# Autodesk Inventor assembly: MG-Grundplatte
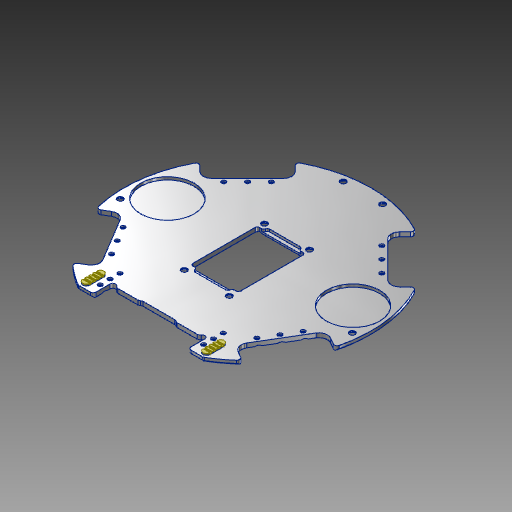
[picture p0: Inventor's stored thumbnail of the model, 512x512]
Saved by Autodesk Inventor 2019.4 (Build 234330000, 330)
## iProperties
Part Number: MG-Grundplatte
Material: Generisch
Document SubType Name: Assembly
Designer: rYan
Mass: 128.652 g
Surface Area: 395.086 cm^2
Volume: 47.6131 cm^3
Density: 2.70203 g/cm^3
Author: rYan
## Documents named in this file (3)
- D:\TIGERsGIT\Hardware\mechanik\2020\Inventor\Robot\MG-Grundplatte.iam
- D:\TIGERsGIT\Hardware\mechanik\2020\Inventor\Robot\Grundplatte.ipt
- D:\TIGERsGIT\Hardware\mechanik\2020\Inventor\Robot\Dribbler\Dribblerdaempfer Unten.ipt
## Components (3 placed, 2 different names)
1. Grundplatte:1 — Fluchtend:1, Passend:1, Passend:2, Passend:3, Passend:4, Tangential:1, Tangential:2, Passend:5, Passend:6
2. Dribblerdaempfer Unten:1 — Passend:3, Tangential:2, Passend:6
3. Dribblerdaempfer Unten:2 — Passend:4, Tangential:1, Passend:5
## Relationships (9: Mate 6, Tangent 2, Flush 1)
- Fluchtend:1 [Flush]: Grundplatte:1
- Passend:1 [Mate]: Grundplatte:1
- Passend:2 [Mate]: Grundplatte:1
- Passend:3 [Mate]: Grundplatte:1 ↔ Dribblerdaempfer Unten:1
- Passend:4 [Mate]: Grundplatte:1 ↔ Dribblerdaempfer Unten:2
- Tangential:1: Grundplatte:1 ↔ Dribblerdaempfer Unten:2
- Tangential:2: Grundplatte:1 ↔ Dribblerdaempfer Unten:1
- Passend:5 [Mate]: Grundplatte:1 ↔ Dribblerdaempfer Unten:2
- Passend:6 [Mate]: Grundplatte:1 ↔ Dribblerdaempfer Unten:1
